# Autodesk Inventor assembly: herramientaParaRobot
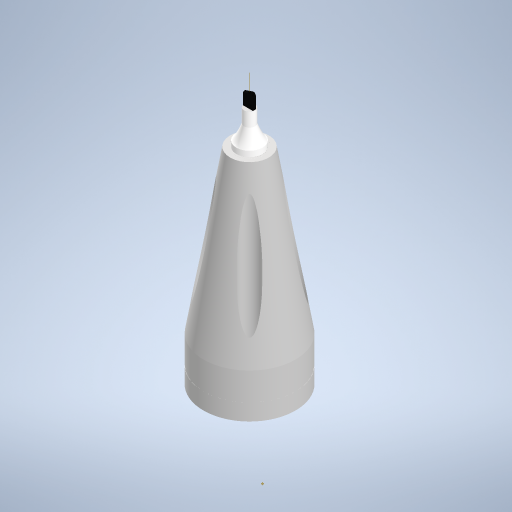
[picture p0: Inventor's stored thumbnail of the model, 512x512]
Saved by Autodesk Inventor 2023 (Build 270158000, 158)
## iProperties
Created: 2022-08-27
Part Number: herramientaParaRobot
Document SubType Name: Assembly
Designer: SAMJ
Author: SAMJ
## Documents named in this file (4)
- D:\Desktop\8 Octavo semestre\Robótica\Lab\Prac1v2\herramientaParaRobot.iam
- D:\Desktop\8 Octavo semestre\Robótica\Lab\Prac1v2\Base.ipt
- D:\Desktop\8 Octavo semestre\Robótica\Lab\Prac1v2\Tapa.ipt
- D:\Desktop\8 Octavo semestre\Robótica\Lab\Prac1\Marcador.ipt
## Components (3 placed, 3 different names)
1. Base:1 — Mate:1, Mate:2, Flush:1, Flush:2, Flush:3
2. Tapa:1 — Mate:1, Mate:2, Mate:3
3. Marcador:1 — Mate:3
## Relationships (6: Mate 3, Flush 3)
- Mate:1: Base:1 ↔ Tapa:1
- Mate:2: Base:1 ↔ Tapa:1
- Mate:3: Tapa:1 ↔ Marcador:1
- Flush:1: Base:1
- Flush:2: Base:1
- Flush:3: Base:1
